# Autodesk Inventor assembly: Ensamble_completo
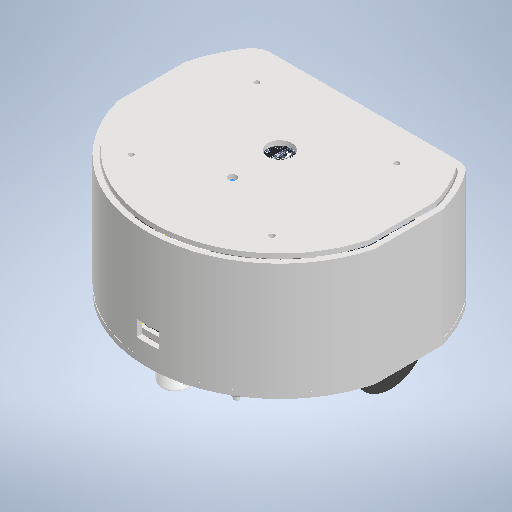
[picture p0: Inventor's stored thumbnail of the model, 512x512]
Saved by Autodesk Inventor 2025.3 (Build 293356030, 356C)
## iProperties
Created: 2025-10-21
Part Number: Ensamble_completo
Document SubType Name: Assembly
Designer: brene
Author: brene
## Documents named in this file (33)
- D:\OneDrive - Estudiantes ITCR\Documentos\GitHub\Atta-Bot-STEM\Chasis\Rediseño_Diego&Carlos\Carcasa 4.0 Rediseño\Ensamble_completo.iam
- D:\OneDrive - Estudiantes ITCR\Documentos\GitHub\Atta-Bot-STEM\Chasis\Rediseño_Diego&Carlos\Carcasa 4.0 Rediseño\base_chasis_v6\base_chasis_v4-dimsAjustadas.ipt
- D:\OneDrive - Estudiantes ITCR\Documentos\GitHub\Atta-Bot-STEM\Chasis\Rediseño_Diego&Carlos\Carcasa 4.0 Rediseño\base_chasis_v6.ipt
- D:\OneDrive - Estudiantes ITCR\Documentos\GitHub\Atta-Bot-STEM\Chasis\Rediseño_Diego&Carlos\Content Center Files\en-US\ISO 4762(2)\ISO 4762 - M2 x 12ISO.ipt
- D:\OneDrive - Estudiantes ITCR\Documentos\GitHub\Atta-Bot-STEM\Chasis\Rediseño_Diego&Carlos\switch.ipt
- D:\OneDrive - Estudiantes ITCR\Documentos\GitHub\Atta-Bot-STEM\Chasis\Rediseño_Diego&Carlos\Content Center Files\en-US\ISO 4762(2)\ISO 4762 - M2 x 8ISO.ipt
- D:\OneDrive - Estudiantes ITCR\Documentos\GitHub\Atta-Bot-STEM\Chasis\Rediseño_Diego&Carlos\Content Center Files\en-US\ISO 4032(2)\ISO 4032 - M2 - ISO.ipt
- D:\OneDrive - Estudiantes ITCR\Documentos\GitHub\Atta-Bot-STEM\Chasis\Rediseño_Diego&Carlos\ball_caster.ipt
- D:\OneDrive - Estudiantes ITCR\Documentos\GitHub\Atta-Bot-STEM\Chasis\Rediseño_Diego&Carlos\sensorInferior.ipt
- D:\OneDrive - Estudiantes ITCR\Documentos\GitHub\Atta-Bot-STEM\Chasis\Rediseño_Diego&Carlos\Content Center Files\en-US\ISO 4762(2)\ISO 4762 - M3 x 12ISO.ipt
- D:\OneDrive - Estudiantes ITCR\Documentos\GitHub\Atta-Bot-STEM\Chasis\Rediseño_Diego&Carlos\Content Center Files\en-US\ISO 4032(2)\ISO 4032 - M3 - ISO.ipt
- D:\OneDrive - Estudiantes ITCR\Documentos\GitHub\Atta-Bot-STEM\Chasis\Rediseño_Diego&Carlos\spacers\hexagonal_spacer_MF_M3_H20_HEX5.5_FTD6_MTL6.ipt
- D:\OneDrive - Estudiantes ITCR\Documentos\GitHub\Atta-Bot-STEM\Chasis\Rediseño_Diego&Carlos\spacers\hexagonal_spacer_MF_M3_H06_HEX5.5_FTD3_MTL6.ipt
- D:\OneDrive - Estudiantes ITCR\Documentos\GitHub\Atta-Bot-STEM\Chasis\Rediseño_Diego&Carlos\Content Center Files\en-US\ISO 4762(2)\ISO 4762 - M3 x 8ISO.ipt
- D:\OneDrive - Estudiantes ITCR\Documentos\GitHub\Atta-Bot-STEM\Chasis\Rediseño_Diego&Carlos\spacers\hexagonal_spacer_MF_M3_H08_HEX5_FTD4_MTL8.ipt
- D:\OneDrive - Estudiantes ITCR\Documentos\GitHub\Atta-Bot-STEM\Chasis\Rediseño_Diego&Carlos\bateria.ipt
- D:\OneDrive - Estudiantes ITCR\Documentos\GitHub\Atta-Bot-STEM\Chasis\Rediseño_Diego&Carlos\base_powerboost.ipt
- D:\OneDrive - Estudiantes ITCR\Documentos\GitHub\Atta-Bot-STEM\Chasis\Rediseño_Diego&Carlos\powerboost.ipt
- D:\OneDrive - Estudiantes ITCR\Documentos\GitHub\Atta-Bot-STEM\Chasis\Rediseño_Diego&Carlos\Carcasa 4.0 Rediseño\base_nivel2_V2.ipt
- D:\OneDrive - Estudiantes ITCR\Documentos\GitHub\Atta-Bot-STEM\Chasis\Rediseño_Diego&Carlos\ideaboard.ipt
- D:\OneDrive - Estudiantes ITCR\Documentos\GitHub\Atta-Bot-STEM\Chasis\Rediseño_Diego&Carlos\sensorFrontal.ipt
- D:\OneDrive - Estudiantes ITCR\Documentos\GitHub\Atta-Bot-STEM\Chasis\Rediseño_Diego&Carlos\Carcasa 4.0 Rediseño\Tower Pro MG90S Micro servo.ipt
- D:\OneDrive - Estudiantes ITCR\Documentos\GitHub\Atta-Bot-STEM\Chasis\Rediseño_Diego&Carlos\spacers\hexagonal_spacer_MF_M3_H10_HEX5.5_FTD6_MTL6.ipt
- D:\OneDrive - Estudiantes ITCR\Documentos\GitHub\Atta-Bot-STEM\Chasis\Rediseño_Diego&Carlos\SoporteMotor_3.0.ipt
- D:\OneDrive - Estudiantes ITCR\Documentos\GitHub\Atta-Bot-STEM\Chasis\Rediseño_Diego&Carlos\motor.ipt
- D:\OneDrive - Estudiantes ITCR\Documentos\GitHub\Atta-Bot-STEM\Chasis\Rediseño_Diego&Carlos\llanta.ipt
- D:\OneDrive - Estudiantes ITCR\Documentos\GitHub\Atta-Bot-STEM\Chasis\Rediseño_Diego&Carlos\Carcasa 4.0 Rediseño\carcasa4.0.ipt
- D:\OneDrive - Estudiantes ITCR\Documentos\GitHub\Atta-Bot-STEM\Chasis\Rediseño_Diego&Carlos\Carcasa 4.0 Rediseño\Unidirectional shoulder.ipt
- D:\OneDrive - Estudiantes ITCR\Documentos\GitHub\Atta-Bot-STEM\Chasis\Rediseño_Diego&Carlos\Carcasa 4.0 Rediseño\SujecionServo.ipt
- D:\OneDrive - Estudiantes ITCR\Documentos\New folder\ISO 4762(2)\ISO 4762 - M3 x 8ISO.ipt
- D:\OneDrive - Estudiantes ITCR\Documentos\New folder\ISO 4032(2)\ISO 4032 - M2,5 - ISO.ipt
- D:\OneDrive - Estudiantes ITCR\Documentos\New folder\ISO 4762(2)\ISO 4762 - M3 x 30ISO.ipt
- D:\OneDrive - Estudiantes ITCR\Documentos\GitHub\Atta-Bot-STEM\Chasis\Rediseño_Diego&Carlos\Carcasa 4.0 Rediseño\tapa_carcasa_4.0_v2.ipt
## Components (107 placed, 30 different names)
1. base_chasis_v4-dimsAjustadas:2 — Mate:1, Mate:2, Mate:4, Mate:6, Insert:1, Insert:2, Mate:7, Tangent:1, Tangent:2, Mate:8, Mate:10, Tangent:3, Tangent:4, Mate:12, Mate:13, Mate:14, Mate:15, Mate:24, Mate:26, Mate:32, Mate:33, Mate:34, Mate:35, Mate:36, Mate:38, Mate:44, Mate:45, Mate:46, Mate:47, Mate:48, Mate:49, Mate:50, Mate:51, Mate:52, Mate:54, Mate:56, Mate:58, Mate:60, Mate:146, Mate:147, Mate:148, Mate:149, Mate:150, Mate:151, Mate:152, Mate:153, Mate:154, Mate:161, Mate:169, Mate:183, Mate:185, Mate:187, Mate:189, Mate:190, Mate:192, Mate:194, Mate:196, Mate:202, Mate:203, Mate:204, Mate:207, Angle:1, Mate:209, Flush:211, Mate:210, Angle:2, Angle:3, Angle:6, Angle:7, Mate:211, Mate:212, Mate:218, Mate:220, Insert:5, Insert:6, Mate:226, Mate:228, Mate:229, Mate:231, Mate:232, Mate:233, Mate:234
2. switch:1 — Mate:1, Mate:2, Mate:3, Mate:5, Angle:3
3. ISO 4762 M2 x 8:1 — Mate:5, Mate:6
4. ISO 4762 M2 x 8:2 — Mate:3, Mate:4
5. ISO 4032 M2:1 — Insert:1
6. ISO 4032 M2:2 — Insert:2
7. ball_caster:1 — Mate:7, Tangent:1, Tangent:2, Mate:9, Mate:11
8. ISO 4762 M2 x 8:3 — Mate:10, Mate:11, Tangent:3
9. ISO 4762 M2 x 8:4 — Mate:8, Mate:9, Tangent:4
10. sensorInferior:1 — Mate:16, Mate:17, Mate:20, Angle:7
11. sensorInferior:2 — Mate:18, Mate:19, Mate:22, Angle:6
12. ISO 4762 M3 x 12:1 — Mate:20, Mate:21, Mate:25
13. ISO 4762 M3 x 12:2 — Mate:22, Mate:23, Mate:27
14. ISO 4032 M3:1 — Mate:12, Mate:13, Mate:16, Mate:17, Mate:21
15. ISO 4032 M3:2 — Mate:14, Mate:15, Mate:18, Mate:19, Mate:23
16. hexagonal_spacer_MF_M3_H20_HEX5.5_FTD6_MTL6:1 — Mate:24, Mate:25, Mate:136, Mate:139
17. hexagonal_spacer_MF_M3_H20_HEX5.5_FTD6_MTL6:2 — Mate:26, Mate:27, Mate:135, Mate:141
18. hexagonal_spacer_MF_M3_H20_HEX5.5_FTD6_MTL6:3 — Mate:38, Mate:39, Mate:143
19. hexagonal_spacer_MF_M3_H20_HEX5.5_FTD6_MTL6:4 — Mate:36, Mate:37, Mate:137, Mate:145
20. ISO 4762 M3 x 8:1 — Mate:32, Mate:33, Mate:37
21. ISO 4762 M3 x 8:2 — Mate:34, Mate:35, Mate:39
22. hexagonal_spacer_MF_M3_H08_HEX5_FTD4_MTL8:1 — Mate:56, Mate:57, Mate:61
23. hexagonal_spacer_MF_M3_H08_HEX5_FTD4_MTL8:2 — Mate:58, Mate:59, Mate:88
24. hexagonal_spacer_MF_M3_H08_HEX5_FTD4_MTL8:3 — Mate:52, Mate:53, Mate:89
25. hexagonal_spacer_MF_M3_H08_HEX5_FTD4_MTL8:4 — Mate:54, Mate:55, Mate:90
26. ISO 4032 M3:3 — Mate:44, Mate:45, Mate:55
27. ISO 4032 M3:4 — Mate:46, Mate:47, Mate:53
28. ISO 4032 M3:5 — Mate:50, Mate:51, Mate:59
29. ISO 4032 M3:6 — Mate:48, Mate:49, Mate:57
30. bateria:1 — Mate:60, Mate:61, Mate:146, Angle:2
31. base_powerboost:1 — Mate:62, Mate:63, Mate:64, Mate:65, Mate:66, Mate:67, Mate:68, Mate:69, Mate:80, Mate:82, Mate:84, Mate:86, Mate:88, Mate:89, Mate:90, Mate:91, Mate:92, Mate:93, Mate:94, Mate:95, Mate:96, Mate:97, Mate:98, Mate:99
32. powerboost:1 — Mate:70, Mate:71, Mate:72, Mate:73, Mate:74, Mate:75, Mate:76, Mate:77, Mate:78, Mate:79
33. ISO 4762 M2 x 12:1 — Mate:74, Mate:75, Mate:81
34. ISO 4762 M2 x 12:2 — Mate:72, Mate:73, Mate:83
35. ISO 4762 M2 x 8:5 — Mate:78, Mate:79, Mate:85
36. ISO 4762 M2 x 8:6 — Mate:76, Mate:77, Mate:87, Mate:91
37. ISO 4032 M2:3 — Mate:68, Mate:69
38. ISO 4032 M2:4 — Mate:62, Mate:63, Mate:71
39. ISO 4032 M2:5 — Mate:66, Mate:67
40. ISO 4032 M2:6 — Mate:64, Mate:65, Mate:70
41. ISO 4032 M2:7 — Mate:82, Mate:83
42. ISO 4032 M2:8 — Mate:86, Mate:87
43. ISO 4032 M2:9 — Mate:80, Mate:81
44. ISO 4032 M2:10 — Mate:84, Mate:85
45. ISO 4762 M3 x 8:3 — Mate:98, Mate:99
46. ISO 4762 M3 x 8:4 — Mate:92, Mate:93
47. ISO 4762 M3 x 8:5 — Mate:96, Mate:97
48. ISO 4762 M3 x 8:6 — Mate:94, Mate:95
49. base_nivel2_V2:1 — Mate:100, Mate:101, Mate:102, Mate:103, Mate:104, Mate:105, Mate:106, Mate:107, Mate:111, Mate:112, Mate:113, Mate:114, Mate:115, Mate:116, Mate:117, Mate:118, Mate:127, Mate:129, Mate:131, Mate:133, Mate:135, Mate:136, Mate:137, Mate:138, Mate:140, Mate:142, Mate:144, Mate:201, Angle:4, Angle:5, Insert:3, Insert:4
50. ideaboard:1 — Mate:108, Mate:109, Mate:110, Mate:174, Mate:176, Mate:178, Mate:180
51. hexagonal_spacer_MF_M3_H06_HEX5.5_FTD3_MTL6:5 — Mate:102, Mate:103, Mate:128, Mate:181
52. hexagonal_spacer_MF_M3_H06_HEX5.5_FTD3_MTL6:6 — Mate:100, Mate:101, Mate:109, Mate:130, Mate:179
53. hexagonal_spacer_MF_M3_H06_HEX5.5_FTD3_MTL6:7 — Mate:106, Mate:107, Mate:134, Mate:177
54. hexagonal_spacer_MF_M3_H06_HEX5.5_FTD3_MTL6:8 — Mate:104, Mate:105, Mate:108, Mate:110, Mate:132, Mate:175
55. hexagonal_spacer_MF_M3_H06_HEX5.5_FTD3_MTL6:9 — Mate:111, Mate:112, Mate:121, Mate:122, Mate:124
56. hexagonal_spacer_MF_M3_H06_HEX5.5_FTD3_MTL6:10 — Mate:115, Mate:116, Mate:119, Mate:120, Mate:126
57. ISO 4032 M3:7 — Mate:125, Mate:126
58. ISO 4032 M3:8 — Mate:123, Mate:124
59. ISO 4762 M3 x 8:7 — Mate:117, Mate:118
60. ISO 4762 M3 x 8:8 — Mate:113, Mate:114
61. sensorFrontal:1 — Mate:121, Mate:122, Mate:123, Angle:5
62. sensorFrontal:2 — Mate:119, Mate:120, Mate:125, Angle:4
63. ISO 4032 M3:9 — Mate:133, Mate:134
64. ISO 4032 M3:10 — Mate:129, Mate:130
65. ISO 4032 M3:11 — Mate:131, Mate:132
66. ISO 4032 M3:12 — Mate:127, Mate:128
67. ISO 4032 M3:13 — Mate:142, Mate:143
68. ISO 4032 M3:14 — Mate:138, Mate:139
69. ISO 4032 M3:15 — Mate:140, Mate:141
70. ISO 4032 M3:16 — Mate:144, Mate:145
71. hexagonal_spacer_MF_M3_H10_HEX5.5_FTD6_MTL6:1 — Mate:147, Mate:149
72. hexagonal_spacer_MF_M3_H10_HEX5.5_FTD6_MTL6:2 — Mate:148, Mate:150
73. ISO 4762 M3 x 8:9 — Mate:153, Mate:154
74. ISO 4762 M3 x 8:10 — Mate:151, Mate:152
75. motor:1 — Mate:161, Mate:163, Mate:164, Mate:227, Tangent:5
76. motor:2 — Mate:169, Mate:171, Mate:172, Mate:230, Tangent:6
77. llanta:1 — Mate:163, Mate:164
78. llanta:2 — Mate:171, Mate:172
79. ISO 4762 M3 x 8:11 — Mate:176, Mate:177
80. ISO 4762 M3 x 8:12 — Mate:180, Mate:181
81. ISO 4762 M3 x 8:13 — Mate:178, Mate:179
82. ISO 4762 M3 x 8:14 — Mate:174, Mate:175
83. ISO 4762 M2 x 8:7 — Mate:185, Mate:195
84. ISO 4762 M2 x 8:8 — Mate:189, Mate:191
85. ISO 4762 M2 x 8:9 — Mate:187, Mate:193
86. ISO 4762 M2 x 8:10 — Mate:183, Mate:197
87. ISO 4032 M2:12 — Mate:190, Mate:191
88. ISO 4032 M2:13 — Mate:192, Mate:193
89. ISO 4032 M2:14 — Mate:196, Mate:197
90. ISO 4032 M2:15 — Mate:194, Mate:195
91. ISO 4762 M3 x 30:3 — Mate:201, Mate:202
92. ISO 4762 M3 x 30:4 — Mate:203, Mate:204
93. Tower Pro MG90S Micro servo:2 — Mate:205, Mate:206, Mate:207, Angle:1, Angle:8, Mate:217, Mate:221
94. Unidirectional shoulder:1 — Mate:205, Mate:206
95. hexagonal_spacer_MF_M3_H10_HEX5.5_FTD6_MTL6:3 — Mate:211, Angle:8, Mate:218, Mate:219
96. hexagonal_spacer_MF_M3_H10_HEX5.5_FTD6_MTL6:4 — Mate:212, Mate:216, Mate:220, Mate:221
97. SujecionServo:1 — Mate:216, Mate:217, Mate:219, Mate:222, Mate:223, Mate:224, Mate:225
98. ISO 4762 M3 x 8:17 — Mate:222, Mate:223
99. ISO 4762 M3 x 8:18 — Mate:224, Mate:225
100. ISO 4032 M2,5:5 — Insert:3
101. ISO 4032 M2,5:6 — Insert:4
102. ISO 4032 M2,5:7 — Insert:5
103. ISO 4032 M2,5:8 — Insert:6
104. SoporteMotor_3.0:1 — Mate:229, Mate:230, Mate:231, Mate:233, Tangent:6
105. SoporteMotor_3.0:2 — Mate:226, Mate:227, Mate:228, Tangent:5, Mate:232
106. carcasa4.0:1 — Mate:234, Mate:235
107. tapa_carcasa_4.0_v2:1 — Mate:235
## Relationships (224: Mate 203, Angle 8, Insert 6, Tangent 6, Flush 1)
- Mate:1: base_chasis_v4-dimsAjustadas:2 ↔ switch:1
- Mate:2: base_chasis_v4-dimsAjustadas:2 ↔ switch:1
- Mate:3: switch:1 ↔ ISO 4762 M2 x 8:2
- Mate:4: base_chasis_v4-dimsAjustadas:2 ↔ ISO 4762 M2 x 8:2
- Mate:5: switch:1 ↔ ISO 4762 M2 x 8:1
- Mate:6: base_chasis_v4-dimsAjustadas:2 ↔ ISO 4762 M2 x 8:1
- Insert:1: base_chasis_v4-dimsAjustadas:2 ↔ ISO 4032 M2:1
- Insert:2: base_chasis_v4-dimsAjustadas:2 ↔ ISO 4032 M2:2
- Mate:7: base_chasis_v4-dimsAjustadas:2 ↔ ball_caster:1
- Tangent:1: base_chasis_v4-dimsAjustadas:2 ↔ ball_caster:1
- Tangent:2: base_chasis_v4-dimsAjustadas:2 ↔ ball_caster:1
- Mate:8: base_chasis_v4-dimsAjustadas:2 ↔ ISO 4762 M2 x 8:4
- Mate:9: ball_caster:1 ↔ ISO 4762 M2 x 8:4
- Mate:10: base_chasis_v4-dimsAjustadas:2 ↔ ISO 4762 M2 x 8:3
- Mate:11: ball_caster:1 ↔ ISO 4762 M2 x 8:3
- Tangent:3: base_chasis_v4-dimsAjustadas:2 ↔ ISO 4762 M2 x 8:3
- Tangent:4: base_chasis_v4-dimsAjustadas:2 ↔ ISO 4762 M2 x 8:4
- Mate:12: base_chasis_v4-dimsAjustadas:2 ↔ ISO 4032 M3:1
- Mate:13: base_chasis_v4-dimsAjustadas:2 ↔ ISO 4032 M3:1
- Mate:14: base_chasis_v4-dimsAjustadas:2 ↔ ISO 4032 M3:2
- Mate:15: base_chasis_v4-dimsAjustadas:2 ↔ ISO 4032 M3:2
- Mate:16: sensorInferior:1 ↔ ISO 4032 M3:1
- Mate:17: sensorInferior:1 ↔ ISO 4032 M3:1
- Mate:18: sensorInferior:2 ↔ ISO 4032 M3:2
- Mate:19: sensorInferior:2 ↔ ISO 4032 M3:2
- Mate:20: sensorInferior:1 ↔ ISO 4762 M3 x 12:1
- Mate:21: ISO 4762 M3 x 12:1 ↔ ISO 4032 M3:1
- Mate:22: sensorInferior:2 ↔ ISO 4762 M3 x 12:2
- Mate:23: ISO 4762 M3 x 12:2 ↔ ISO 4032 M3:2
- Mate:24: base_chasis_v4-dimsAjustadas:2 ↔ hexagonal_spacer_MF_M3_H20_HEX5.5_FTD6_MTL6:1
- Mate:25: ISO 4762 M3 x 12:1 ↔ hexagonal_spacer_MF_M3_H20_HEX5.5_FTD6_MTL6:1
- Mate:26: base_chasis_v4-dimsAjustadas:2 ↔ hexagonal_spacer_MF_M3_H20_HEX5.5_FTD6_MTL6:2
- Mate:27: ISO 4762 M3 x 12:2 ↔ hexagonal_spacer_MF_M3_H20_HEX5.5_FTD6_MTL6:2
- Mate:32: base_chasis_v4-dimsAjustadas:2 ↔ ISO 4762 M3 x 8:1
- Mate:33: base_chasis_v4-dimsAjustadas:2 ↔ ISO 4762 M3 x 8:1
- Mate:34: base_chasis_v4-dimsAjustadas:2 ↔ ISO 4762 M3 x 8:2
- Mate:35: base_chasis_v4-dimsAjustadas:2 ↔ ISO 4762 M3 x 8:2
- Mate:36: base_chasis_v4-dimsAjustadas:2 ↔ hexagonal_spacer_MF_M3_H20_HEX5.5_FTD6_MTL6:4
- Mate:37: hexagonal_spacer_MF_M3_H20_HEX5.5_FTD6_MTL6:4 ↔ ISO 4762 M3 x 8:1
- Mate:38: base_chasis_v4-dimsAjustadas:2 ↔ hexagonal_spacer_MF_M3_H20_HEX5.5_FTD6_MTL6:3
- Mate:39: hexagonal_spacer_MF_M3_H20_HEX5.5_FTD6_MTL6:3 ↔ ISO 4762 M3 x 8:2
- Mate:44: base_chasis_v4-dimsAjustadas:2 ↔ ISO 4032 M3:3
- Mate:45: base_chasis_v4-dimsAjustadas:2 ↔ ISO 4032 M3:3
- Mate:46: base_chasis_v4-dimsAjustadas:2 ↔ ISO 4032 M3:4
- Mate:47: base_chasis_v4-dimsAjustadas:2 ↔ ISO 4032 M3:4
- Mate:48: base_chasis_v4-dimsAjustadas:2 ↔ ISO 4032 M3:6
- Mate:49: base_chasis_v4-dimsAjustadas:2 ↔ ISO 4032 M3:6
- Mate:50: base_chasis_v4-dimsAjustadas:2 ↔ ISO 4032 M3:5
- Mate:51: base_chasis_v4-dimsAjustadas:2 ↔ ISO 4032 M3:5
- Mate:52: base_chasis_v4-dimsAjustadas:2 ↔ hexagonal_spacer_MF_M3_H08_HEX5_FTD4_MTL8:3
- Mate:53: hexagonal_spacer_MF_M3_H08_HEX5_FTD4_MTL8:3 ↔ ISO 4032 M3:4
- Mate:54: base_chasis_v4-dimsAjustadas:2 ↔ hexagonal_spacer_MF_M3_H08_HEX5_FTD4_MTL8:4
- Mate:55: hexagonal_spacer_MF_M3_H08_HEX5_FTD4_MTL8:4 ↔ ISO 4032 M3:3
- Mate:56: base_chasis_v4-dimsAjustadas:2 ↔ hexagonal_spacer_MF_M3_H08_HEX5_FTD4_MTL8:1
- Mate:57: hexagonal_spacer_MF_M3_H08_HEX5_FTD4_MTL8:1 ↔ ISO 4032 M3:6
- Mate:58: base_chasis_v4-dimsAjustadas:2 ↔ hexagonal_spacer_MF_M3_H08_HEX5_FTD4_MTL8:2
- Mate:59: hexagonal_spacer_MF_M3_H08_HEX5_FTD4_MTL8:2 ↔ ISO 4032 M3:5
- Mate:60: base_chasis_v4-dimsAjustadas:2 ↔ bateria:1
- Mate:61: hexagonal_spacer_MF_M3_H08_HEX5_FTD4_MTL8:1 ↔ bateria:1
- Mate:62: base_powerboost:1 ↔ ISO 4032 M2:4
- Mate:63: base_powerboost:1 ↔ ISO 4032 M2:4
- Mate:64: base_powerboost:1 ↔ ISO 4032 M2:6
- Mate:65: base_powerboost:1 ↔ ISO 4032 M2:6
- Mate:66: base_powerboost:1 ↔ ISO 4032 M2:5
- Mate:67: base_powerboost:1 ↔ ISO 4032 M2:5
- Mate:68: base_powerboost:1 ↔ ISO 4032 M2:3
- Mate:69: base_powerboost:1 ↔ ISO 4032 M2:3
- Mate:70: powerboost:1 ↔ ISO 4032 M2:6
- Mate:71: powerboost:1 ↔ ISO 4032 M2:4
- Mate:72: powerboost:1 ↔ ISO 4762 M2 x 12:2
- Mate:73: powerboost:1 ↔ ISO 4762 M2 x 12:2
- Mate:74: powerboost:1 ↔ ISO 4762 M2 x 12:1
- Mate:75: powerboost:1 ↔ ISO 4762 M2 x 12:1
- Mate:76: powerboost:1 ↔ ISO 4762 M2 x 8:6
- Mate:77: powerboost:1 ↔ ISO 4762 M2 x 8:6
- Mate:78: powerboost:1 ↔ ISO 4762 M2 x 8:5
- Mate:79: powerboost:1 ↔ ISO 4762 M2 x 8:5
- Mate:80: base_powerboost:1 ↔ ISO 4032 M2:9
- Mate:81: ISO 4762 M2 x 12:1 ↔ ISO 4032 M2:9
- Mate:82: base_powerboost:1 ↔ ISO 4032 M2:7
- Mate:83: ISO 4762 M2 x 12:2 ↔ ISO 4032 M2:7
- Mate:84: base_powerboost:1 ↔ ISO 4032 M2:10
- Mate:85: ISO 4762 M2 x 8:5 ↔ ISO 4032 M2:10
- Mate:86: base_powerboost:1 ↔ ISO 4032 M2:8
- Mate:87: ISO 4762 M2 x 8:6 ↔ ISO 4032 M2:8
- Mate:88: hexagonal_spacer_MF_M3_H08_HEX5_FTD4_MTL8:2 ↔ base_powerboost:1
- Mate:89: hexagonal_spacer_MF_M3_H08_HEX5_FTD4_MTL8:3 ↔ base_powerboost:1
- Mate:90: hexagonal_spacer_MF_M3_H08_HEX5_FTD4_MTL8:4 ↔ base_powerboost:1
- Mate:91: base_powerboost:1 ↔ ISO 4762 M2 x 8:6
- Mate:92: base_powerboost:1 ↔ ISO 4762 M3 x 8:4
- Mate:93: base_powerboost:1 ↔ ISO 4762 M3 x 8:4
- Mate:94: base_powerboost:1 ↔ ISO 4762 M3 x 8:6
- Mate:95: base_powerboost:1 ↔ ISO 4762 M3 x 8:6
- Mate:96: base_powerboost:1 ↔ ISO 4762 M3 x 8:5
- Mate:97: base_powerboost:1 ↔ ISO 4762 M3 x 8:5
- Mate:98: base_powerboost:1 ↔ ISO 4762 M3 x 8:3
- Mate:99: base_powerboost:1 ↔ ISO 4762 M3 x 8:3
- Mate:100: base_nivel2_V2:1 ↔ hexagonal_spacer_MF_M3_H06_HEX5.5_FTD3_MTL6:6
- Mate:101: base_nivel2_V2:1 ↔ hexagonal_spacer_MF_M3_H06_HEX5.5_FTD3_MTL6:6
- Mate:102: base_nivel2_V2:1 ↔ hexagonal_spacer_MF_M3_H06_HEX5.5_FTD3_MTL6:5
- Mate:103: base_nivel2_V2:1 ↔ hexagonal_spacer_MF_M3_H06_HEX5.5_FTD3_MTL6:5
- Mate:104: base_nivel2_V2:1 ↔ hexagonal_spacer_MF_M3_H06_HEX5.5_FTD3_MTL6:8
- Mate:105: base_nivel2_V2:1 ↔ hexagonal_spacer_MF_M3_H06_HEX5.5_FTD3_MTL6:8
- Mate:106: base_nivel2_V2:1 ↔ hexagonal_spacer_MF_M3_H06_HEX5.5_FTD3_MTL6:7
- Mate:107: base_nivel2_V2:1 ↔ hexagonal_spacer_MF_M3_H06_HEX5.5_FTD3_MTL6:7
- Mate:108: ideaboard:1 ↔ hexagonal_spacer_MF_M3_H06_HEX5.5_FTD3_MTL6:8
- Mate:109: ideaboard:1 ↔ hexagonal_spacer_MF_M3_H06_HEX5.5_FTD3_MTL6:6
- Mate:110: ideaboard:1 ↔ hexagonal_spacer_MF_M3_H06_HEX5.5_FTD3_MTL6:8
- Mate:111: base_nivel2_V2:1 ↔ hexagonal_spacer_MF_M3_H06_HEX5.5_FTD3_MTL6:9
- Mate:112: base_nivel2_V2:1 ↔ hexagonal_spacer_MF_M3_H06_HEX5.5_FTD3_MTL6:9
- Mate:113: base_nivel2_V2:1 ↔ ISO 4762 M3 x 8:8
- Mate:114: base_nivel2_V2:1 ↔ ISO 4762 M3 x 8:8
- Mate:115: base_nivel2_V2:1 ↔ hexagonal_spacer_MF_M3_H06_HEX5.5_FTD3_MTL6:10
- Mate:116: base_nivel2_V2:1 ↔ hexagonal_spacer_MF_M3_H06_HEX5.5_FTD3_MTL6:10
- Mate:117: base_nivel2_V2:1 ↔ ISO 4762 M3 x 8:7
- Mate:118: base_nivel2_V2:1 ↔ ISO 4762 M3 x 8:7
- Mate:119: hexagonal_spacer_MF_M3_H06_HEX5.5_FTD3_MTL6:10 ↔ sensorFrontal:2
- Mate:120: hexagonal_spacer_MF_M3_H06_HEX5.5_FTD3_MTL6:10 ↔ sensorFrontal:2
- Mate:121: hexagonal_spacer_MF_M3_H06_HEX5.5_FTD3_MTL6:9 ↔ sensorFrontal:1
- Mate:122: hexagonal_spacer_MF_M3_H06_HEX5.5_FTD3_MTL6:9 ↔ sensorFrontal:1
- Mate:123: ISO 4032 M3:8 ↔ sensorFrontal:1
- Mate:124: hexagonal_spacer_MF_M3_H06_HEX5.5_FTD3_MTL6:9 ↔ ISO 4032 M3:8
- Mate:125: ISO 4032 M3:7 ↔ sensorFrontal:2
- Mate:126: hexagonal_spacer_MF_M3_H06_HEX5.5_FTD3_MTL6:10 ↔ ISO 4032 M3:7
- Mate:127: base_nivel2_V2:1 ↔ ISO 4032 M3:12
- Mate:128: hexagonal_spacer_MF_M3_H06_HEX5.5_FTD3_MTL6:5 ↔ ISO 4032 M3:12
- Mate:129: base_nivel2_V2:1 ↔ ISO 4032 M3:10
- Mate:130: hexagonal_spacer_MF_M3_H06_HEX5.5_FTD3_MTL6:6 ↔ ISO 4032 M3:10
- Mate:131: base_nivel2_V2:1 ↔ ISO 4032 M3:11
- Mate:132: hexagonal_spacer_MF_M3_H06_HEX5.5_FTD3_MTL6:8 ↔ ISO 4032 M3:11
- Mate:133: base_nivel2_V2:1 ↔ ISO 4032 M3:9
- Mate:134: hexagonal_spacer_MF_M3_H06_HEX5.5_FTD3_MTL6:7 ↔ ISO 4032 M3:9
- Mate:135: hexagonal_spacer_MF_M3_H20_HEX5.5_FTD6_MTL6:2 ↔ base_nivel2_V2:1
- Mate:136: hexagonal_spacer_MF_M3_H20_HEX5.5_FTD6_MTL6:1 ↔ base_nivel2_V2:1
- Mate:137: hexagonal_spacer_MF_M3_H20_HEX5.5_FTD6_MTL6:4 ↔ base_nivel2_V2:1
- Mate:138: base_nivel2_V2:1 ↔ ISO 4032 M3:14
- Mate:139: hexagonal_spacer_MF_M3_H20_HEX5.5_FTD6_MTL6:1 ↔ ISO 4032 M3:14
- Mate:140: base_nivel2_V2:1 ↔ ISO 4032 M3:15
- Mate:141: hexagonal_spacer_MF_M3_H20_HEX5.5_FTD6_MTL6:2 ↔ ISO 4032 M3:15
- Mate:142: base_nivel2_V2:1 ↔ ISO 4032 M3:13
- Mate:143: hexagonal_spacer_MF_M3_H20_HEX5.5_FTD6_MTL6:3 ↔ ISO 4032 M3:13
- Mate:144: base_nivel2_V2:1 ↔ ISO 4032 M3:16
- Mate:145: hexagonal_spacer_MF_M3_H20_HEX5.5_FTD6_MTL6:4 ↔ ISO 4032 M3:16
- Mate:146: base_chasis_v4-dimsAjustadas:2 ↔ bateria:1
- Mate:147: base_chasis_v4-dimsAjustadas:2 ↔ hexagonal_spacer_MF_M3_H10_HEX5.5_FTD6_MTL6:1
- Mate:148: base_chasis_v4-dimsAjustadas:2 ↔ hexagonal_spacer_MF_M3_H10_HEX5.5_FTD6_MTL6:2
- Mate:149: base_chasis_v4-dimsAjustadas:2 ↔ hexagonal_spacer_MF_M3_H10_HEX5.5_FTD6_MTL6:1
- Mate:150: base_chasis_v4-dimsAjustadas:2 ↔ hexagonal_spacer_MF_M3_H10_HEX5.5_FTD6_MTL6:2
- Mate:151: base_chasis_v4-dimsAjustadas:2 ↔ ISO 4762 M3 x 8:10
- Mate:152: base_chasis_v4-dimsAjustadas:2 ↔ ISO 4762 M3 x 8:10
- Mate:153: base_chasis_v4-dimsAjustadas:2 ↔ ISO 4762 M3 x 8:9
- Mate:154: base_chasis_v4-dimsAjustadas:2 ↔ ISO 4762 M3 x 8:9
- Mate:161: base_chasis_v4-dimsAjustadas:2 ↔ motor:1
- Mate:163: motor:1 ↔ llanta:1
- Mate:164: motor:1 ↔ llanta:1
- Mate:169: base_chasis_v4-dimsAjustadas:2 ↔ motor:2
- Mate:171: motor:2 ↔ llanta:2
- Mate:172: motor:2 ↔ llanta:2
- Mate:174: ideaboard:1 ↔ ISO 4762 M3 x 8:14
- Mate:175: hexagonal_spacer_MF_M3_H06_HEX5.5_FTD3_MTL6:8 ↔ ISO 4762 M3 x 8:14
- Mate:176: ideaboard:1 ↔ ISO 4762 M3 x 8:11
- Mate:177: hexagonal_spacer_MF_M3_H06_HEX5.5_FTD3_MTL6:7 ↔ ISO 4762 M3 x 8:11
- Mate:178: ideaboard:1 ↔ ISO 4762 M3 x 8:13
- Mate:179: hexagonal_spacer_MF_M3_H06_HEX5.5_FTD3_MTL6:6 ↔ ISO 4762 M3 x 8:13
- Mate:180: ideaboard:1 ↔ ISO 4762 M3 x 8:12
- Mate:181: hexagonal_spacer_MF_M3_H06_HEX5.5_FTD3_MTL6:5 ↔ ISO 4762 M3 x 8:12
- Mate:183: base_chasis_v4-dimsAjustadas:2 ↔ ISO 4762 M2 x 8:10
- Mate:185: base_chasis_v4-dimsAjustadas:2 ↔ ISO 4762 M2 x 8:7
- Mate:187: base_chasis_v4-dimsAjustadas:2 ↔ ISO 4762 M2 x 8:9
- Mate:189: base_chasis_v4-dimsAjustadas:2 ↔ ISO 4762 M2 x 8:8
- Mate:190: base_chasis_v4-dimsAjustadas:2 ↔ ISO 4032 M2:12
- Mate:191: ISO 4762 M2 x 8:8 ↔ ISO 4032 M2:12
- Mate:192: base_chasis_v4-dimsAjustadas:2 ↔ ISO 4032 M2:13
- Mate:193: ISO 4762 M2 x 8:9 ↔ ISO 4032 M2:13
- Mate:194: base_chasis_v4-dimsAjustadas:2 ↔ ISO 4032 M2:15
- Mate:195: ISO 4762 M2 x 8:7 ↔ ISO 4032 M2:15
- Mate:196: base_chasis_v4-dimsAjustadas:2 ↔ ISO 4032 M2:14
- Mate:197: ISO 4762 M2 x 8:10 ↔ ISO 4032 M2:14
- Mate:201: base_nivel2_V2:1 ↔ ISO 4762 M3 x 30:3
- Mate:202: base_chasis_v4-dimsAjustadas:2 ↔ ISO 4762 M3 x 30:3
- Mate:203: base_chasis_v4-dimsAjustadas:2 ↔ ISO 4762 M3 x 30:4
- Mate:204: base_chasis_v4-dimsAjustadas:2 ↔ ISO 4762 M3 x 30:4
- Mate:205: Tower Pro MG90S Micro servo:2 ↔ Unidirectional shoulder:1
- Mate:206 (1 mm): Tower Pro MG90S Micro servo:2 ↔ Unidirectional shoulder:1
- Mate:207: base_chasis_v4-dimsAjustadas:2 ↔ Tower Pro MG90S Micro servo:2
- Angle:1 (0 deg): base_chasis_v4-dimsAjustadas:2 ↔ Tower Pro MG90S Micro servo:2
- Mate:209: base_chasis_v4-dimsAjustadas:2
- Flush:211: base_chasis_v4-dimsAjustadas:2
- Mate:210: base_chasis_v4-dimsAjustadas:2
- Angle:2 (0 deg): base_chasis_v4-dimsAjustadas:2 ↔ bateria:1
- Angle:3 (180 deg): base_chasis_v4-dimsAjustadas:2 ↔ switch:1
- Angle:4 (180 deg): base_nivel2_V2:1 ↔ sensorFrontal:2
- Angle:5 (180 deg): base_nivel2_V2:1 ↔ sensorFrontal:1
- Angle:6 (180 deg): base_chasis_v4-dimsAjustadas:2 ↔ sensorInferior:2
- Angle:7 (180 deg): base_chasis_v4-dimsAjustadas:2 ↔ sensorInferior:1
- Mate:211: base_chasis_v4-dimsAjustadas:2 ↔ hexagonal_spacer_MF_M3_H10_HEX5.5_FTD6_MTL6:3
- Mate:212: base_chasis_v4-dimsAjustadas:2 ↔ hexagonal_spacer_MF_M3_H10_HEX5.5_FTD6_MTL6:4
- Angle:8 (-90 deg): Tower Pro MG90S Micro servo:2 ↔ hexagonal_spacer_MF_M3_H10_HEX5.5_FTD6_MTL6:3
- Mate:216: hexagonal_spacer_MF_M3_H10_HEX5.5_FTD6_MTL6:4 ↔ SujecionServo:1
- Mate:217: Tower Pro MG90S Micro servo:2 ↔ SujecionServo:1
- Mate:218: base_chasis_v4-dimsAjustadas:2 ↔ hexagonal_spacer_MF_M3_H10_HEX5.5_FTD6_MTL6:3
- Mate:219: hexagonal_spacer_MF_M3_H10_HEX5.5_FTD6_MTL6:3 ↔ SujecionServo:1
- Mate:220: base_chasis_v4-dimsAjustadas:2 ↔ hexagonal_spacer_MF_M3_H10_HEX5.5_FTD6_MTL6:4
- Mate:221: Tower Pro MG90S Micro servo:2 ↔ hexagonal_spacer_MF_M3_H10_HEX5.5_FTD6_MTL6:4
- Mate:222: SujecionServo:1 ↔ ISO 4762 M3 x 8:17
- Mate:223: SujecionServo:1 ↔ ISO 4762 M3 x 8:17
- Mate:224: SujecionServo:1 ↔ ISO 4762 M3 x 8:18
- Mate:225: SujecionServo:1 ↔ ISO 4762 M3 x 8:18
- Insert:3: base_nivel2_V2:1 ↔ ISO 4032 M2,5:5
- Insert:4: base_nivel2_V2:1 ↔ ISO 4032 M2,5:6
- Insert:5: base_chasis_v4-dimsAjustadas:2 ↔ ISO 4032 M2,5:7
- Insert:6: base_chasis_v4-dimsAjustadas:2 ↔ ISO 4032 M2,5:8
- Mate:226: base_chasis_v4-dimsAjustadas:2 ↔ SoporteMotor_3.0:2
- Mate:227: motor:1 ↔ SoporteMotor_3.0:2
- Mate:228: base_chasis_v4-dimsAjustadas:2 ↔ SoporteMotor_3.0:2
- Mate:229: base_chasis_v4-dimsAjustadas:2 ↔ SoporteMotor_3.0:1
- Mate:230: motor:2 ↔ SoporteMotor_3.0:1
- Mate:231: base_chasis_v4-dimsAjustadas:2 ↔ SoporteMotor_3.0:1
- Tangent:5: motor:1 ↔ SoporteMotor_3.0:2
- Mate:232: base_chasis_v4-dimsAjustadas:2 ↔ SoporteMotor_3.0:2
- Mate:233: base_chasis_v4-dimsAjustadas:2 ↔ SoporteMotor_3.0:1
- Tangent:6: motor:2 ↔ SoporteMotor_3.0:1
- Mate:234: base_chasis_v4-dimsAjustadas:2 ↔ carcasa4.0:1
- Mate:235: carcasa4.0:1 ↔ tapa_carcasa_4.0_v2:1
